# Autodesk Inventor assembly: ground_support
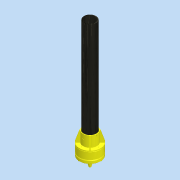
[picture p0: Inventor's stored thumbnail of the model, 180x180]
Saved by Autodesk Inventor 2022 (Build 260153000, 153)
## iProperties
Created: 2021-07-12
Part Number: ground_support
Document SubType Name: Assembly
Designer: nnico
Author: nnico
## Documents named in this file (6)
- C:\Users\nnico\Documents\Desminado Humanitario\Repositories\gpr20_ground_support\assemblies\ground_support.iam
- C:\Users\nnico\Documents\Desminado Humanitario\Repositories\gpr20_ground_support\assemblies\misc\2inx50cm_pipe.ipt
- C:\Users\nnico\Documents\Desminado Humanitario\Repositories\gpr20_ground_support\ipt\ground_support_0.ipt
- C:\Users\nnico\Documents\Desminado Humanitario\Repositories\gpr20_ground_support\ipt\ground_support_1.ipt
- C:\Users\nnico\Documents\Desminado Humanitario\Repositories\gpr20_ground_support\ipt\ground_support_2.ipt
- C:\Users\nnico\Documents\Desminado Humanitario\Repositories\gpr20_ground_support\ipt\ground_support_3.ipt
## Components (5 placed, 5 different names)
1. 2inx50cm_pipe:1 — Rigid:4
2. ground_support_0:1 — Mate:1, Mate:2
3. ground_support_1:1 — Rigid:5, Rigid:6, Mate:1, Mate:2
4. ground_support_2:1 — Rigid:5
5. ground_support_3:1 — Rigid:4, Rigid:6
## Relationships (5: WeldJoint 3, Mate 2)
- Rigid:4 [WeldJoint]: 2inx50cm_pipe:1 ↔ ground_support_3:1
- Rigid:5 [WeldJoint]: ground_support_1:1 ↔ ground_support_2:1
- Rigid:6 [WeldJoint]: ground_support_1:1 ↔ ground_support_3:1
- Mate:1: ground_support_0:1 ↔ ground_support_1:1
- Mate:2: ground_support_0:1 ↔ ground_support_1:1
